# Autodesk Inventor assembly: !Clamp
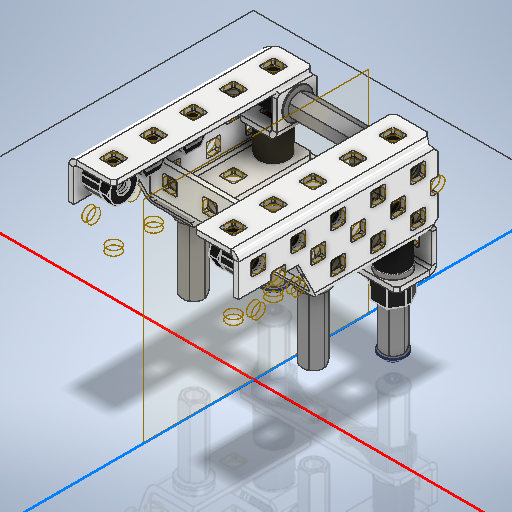
[picture p0: Inventor's stored thumbnail of the model, 512x512]
Saved by Autodesk Inventor 2026 (Build 300175000, 175)
## iProperties
Created: 2025-04-05
Part Number: !Clamp
Document SubType Name: Assembly
Designer: avere
Author: avere
## Documents named in this file (22)
- C:\Users\avere\OneDrive\Documents\VEX-CAD\V5-CAD\Clamp\!Clamp.iam
- C:\Users\avere\OneDrive\Documents\VEX-CAD\VEX-CAD-Inventor\Structure\C Channel\Aluminum 1x2x1\Alu C 1x2x1x5.ipt
- C:\Users\avere\OneDrive\Documents\VEX-CAD\VEX-CAD-Inventor\Motion\Shaft LS\Bearing Flat Low Profile.ipt
- C:\Users\avere\OneDrive\Documents\VEX-CAD\VEX-CAD-Inventor\Structure\Hardware\Nut Nylon\Nut Nylon - Black.ipt
- C:\Users\avere\OneDrive\Documents\VEX-CAD\VEX-CAD-Inventor\Structure\Hardware\Nut Nylon.ipt
- C:\Users\avere\OneDrive\Documents\VEX-CAD\VEX-CAD-Inventor\Structure\Standoff\Standoff .875.ipt
- C:\Users\avere\OneDrive\Documents\VEX-CAD\VEX-CAD-Inventor\Structure\Standoff.ipt
- C:\Users\avere\OneDrive\Documents\VEX-CAD\VEX-CAD-Inventor\Motion\Spacers\Spacer Nylon .375 OD\NSpacer .375 OD x .375.ipt
- C:\Users\avere\OneDrive\Documents\VEX-CAD\VEX-CAD-Inventor\Motion\Spacers\Spacer Nylon .375 OD.ipt
- C:\Users\avere\OneDrive\Documents\VEX-CAD\VEX-CAD-Inventor\Motion\Spacers\Washer Steel\SWasher .375 OD x .062500.ipt
- C:\Users\avere\OneDrive\Documents\VEX-CAD\VEX-CAD-Inventor\Motion\Spacers\Washer Steel.ipt
- C:\Users\avere\OneDrive\Documents\VEX-CAD\VEX-CAD-Inventor\Motion\Spacers\Washer Steel\SWasher .375 OD x .031250.ipt
- C:\Users\avere\OneDrive\Documents\VEX-CAD\VEX-CAD-Inventor\Structure\1-Post Standoff Retainer.ipt
- C:\Users\avere\OneDrive\Documents\VEX-CAD\VEX-CAD-Inventor\Structure\Standoff\Standoff .75.ipt
- C:\Users\avere\OneDrive\Documents\VEX-CAD\VEX-CAD-Inventor\Structure\Hardware\Screw Steel - Star\SScrew Star Smooth .250.ipt
- C:\Users\avere\OneDrive\Documents\VEX-CAD\VEX-CAD-Inventor\Structure\Hardware\Screw Steel - Star.ipt
- C:\Users\avere\OneDrive\Documents\VEX-CAD\VEX-CAD-Inventor\Structure\Angle\Aluminum 1x1\Alu Angle 1x1x1.ipt
- C:\Users\avere\OneDrive\Documents\VEX-CAD\VEX-CAD-Inventor\Motion\Spacers\Washer Steel\SWasher .375 OD x .015625.ipt
- C:\Users\avere\OneDrive\Documents\VEX-CAD\VEX-CAD-Inventor\Motion\Spacers\Washer Teflon\TWasher .375 OD x .04000.ipt
- C:\Users\avere\OneDrive\Documents\VEX-CAD\VEX-CAD-Inventor\Motion\Spacers\Washer Teflon.ipt
- C:\Users\avere\OneDrive\Documents\VEX-CAD\VEX-CAD-Inventor\Structure\C Channel\Aluminum 1x2x1\Alu C 1x2x1x5 Mirrored.ipt
- C:\Users\avere\OneDrive\Documents\VEX-CAD\VEX-CAD-Inventor\Structure\Angle\Aluminum 1x1\Alu Angle 1x1x4.ipt
## Components (41 placed, 15 different names)
1. Alu C 1x2x1x5:1 — Flush:1, Mate:1, Flush:2, Insert:1, Mate:2, Insert:5, Insert:8, Mate:3, Mate:4, Insert:13, Insert:37
2. Bearing Flat Low Profile:1 — Insert:1, Mate:2, Insert:2
3. Nut Nylon - Black:1 — Insert:2
4. Standoff .875:1 — Insert:7
5. NSpacer .375 OD x .375:1 — Insert:4, Insert:5
6. SWasher .375 OD x .062500:1 — Insert:4, Insert:9, Insert:36
7. SWasher .375 OD x .031250:2 — Insert:6, Insert:7
8. SWasher .375 OD x .062500:3 — Insert:6, Insert:8
9. 1-Post Standoff Retainer:1 — Insert:9, Insert:11
10. Standoff .75:2 — Insert:10, Insert:11
11. SScrew Star Smooth .250:1 — Insert:10
12. Alu Angle 1x1x1:1 — Mate:3, Mate:4, Insert:17
13. NSpacer .375 OD x .375:2 — Insert:12, Insert:13
14. SWasher .375 OD x .015625:4 — Insert:12
15. NSpacer .375 OD x .375:3 — Insert:16, Insert:17
16. TWasher .375 OD x .04000:1 — Insert:14, Insert:15
17. TWasher .375 OD x .04000:2 — Insert:14, Insert:16
18. SWasher .375 OD x .031250:5 — Insert:15
19. Alu C 1x2x1x5 Mirrored:1 — Flush:3, Mate:5, Flush:4, Mate:6, Insert:19, Insert:21, Insert:24, Mate:7, Mate:8, Insert:29, Mate:10
20. Bearing Flat Low Profile:2 — Mate:6, Insert:19, Insert:20
21. Nut Nylon - Black:2 — Insert:20
22. Standoff .875:3 — Insert:23
23. NSpacer .375 OD x .375:4 — Insert:21, Insert:22
24. SWasher .375 OD x .062500:6 — Insert:22, Insert:26, Mate:9
25. SWasher .375 OD x .031250:7 — Insert:23, Insert:25
26. SWasher .375 OD x .062500:8 — Insert:24, Insert:25
27. 1-Post Standoff Retainer:2 — Insert:26, Insert:27
28. Standoff .75:4 — Insert:27, Insert:28
29. SScrew Star Smooth .250:2 — Insert:28
30. Alu Angle 1x1x1:2 — Mate:7, Mate:8, Insert:31, Insert:40
31. NSpacer .375 OD x .375:5 — Insert:29, Insert:30
32. SWasher .375 OD x .015625:9 — Insert:30
33. NSpacer .375 OD x .375:6 — Insert:31, Insert:32
34. TWasher .375 OD x .04000:3 — Insert:33, Insert:34
35. TWasher .375 OD x .04000:4 — Insert:32, Insert:33
36. SWasher .375 OD x .031250:10 — Insert:34
37. Alu Angle 1x1x4:1 — Insert:36, Mate:9
38. Alu Angle 1x1x4:2 — Insert:37, Mate:10
39. Standoff .875:5 — Insert:38, Insert:39
40. SWasher .375 OD x .015625:11 — Insert:39
41. SWasher .375 OD x .015625:12 — Insert:38, Insert:40
## Relationships (51: Insert 37, Mate 10, Flush 4)
- Flush:1 (-31.75 mm): Alu C 1x2x1x5:1
- Mate:1 (19.05 mm): Alu C 1x2x1x5:1
- Flush:2 (-12.7 mm): Alu C 1x2x1x5:1
- Insert:1: Alu C 1x2x1x5:1 ↔ Bearing Flat Low Profile:1
- Mate:2: Alu C 1x2x1x5:1 ↔ Bearing Flat Low Profile:1
- Insert:2 (1.27 mm): Bearing Flat Low Profile:1 ↔ Nut Nylon - Black:1
- Insert:4: NSpacer .375 OD x .375:1 ↔ SWasher .375 OD x .062500:1
- Insert:5: Alu C 1x2x1x5:1 ↔ NSpacer .375 OD x .375:1
- Insert:6: SWasher .375 OD x .031250:2 ↔ SWasher .375 OD x .062500:3
- Insert:7: Standoff .875:1 ↔ SWasher .375 OD x .031250:2
- Insert:8: Alu C 1x2x1x5:1 ↔ SWasher .375 OD x .062500:3
- Insert:9 (1.5875 mm): SWasher .375 OD x .062500:1 ↔ 1-Post Standoff Retainer:1
- Insert:10: Standoff .75:2 ↔ SScrew Star Smooth .250:1
- Insert:11: 1-Post Standoff Retainer:1 ↔ Standoff .75:2
- Mate:3: Alu C 1x2x1x5:1 ↔ Alu Angle 1x1x1:1
- Mate:4: Alu C 1x2x1x5:1 ↔ Alu Angle 1x1x1:1
- Insert:12: NSpacer .375 OD x .375:2 ↔ SWasher .375 OD x .015625:4
- Insert:13: Alu C 1x2x1x5:1 ↔ NSpacer .375 OD x .375:2
- Insert:14: TWasher .375 OD x .04000:1 ↔ TWasher .375 OD x .04000:2
- Insert:15: TWasher .375 OD x .04000:1 ↔ SWasher .375 OD x .031250:5
- Insert:16: NSpacer .375 OD x .375:3 ↔ TWasher .375 OD x .04000:2
- Insert:17: Alu Angle 1x1x1:1 ↔ NSpacer .375 OD x .375:3
- Flush:3 (-12.7 mm): Alu C 1x2x1x5 Mirrored:1
- Mate:5 (-19.05 mm): Alu C 1x2x1x5 Mirrored:1
- Flush:4 (-31.75 mm): Alu C 1x2x1x5 Mirrored:1
- Mate:6: Alu C 1x2x1x5 Mirrored:1 ↔ Bearing Flat Low Profile:2
- Insert:19: Alu C 1x2x1x5 Mirrored:1 ↔ Bearing Flat Low Profile:2
- Insert:20 (1.27 mm): Bearing Flat Low Profile:2 ↔ Nut Nylon - Black:2
- Insert:21: Alu C 1x2x1x5 Mirrored:1 ↔ NSpacer .375 OD x .375:4
- Insert:22: NSpacer .375 OD x .375:4 ↔ SWasher .375 OD x .062500:6
- Insert:23: Standoff .875:3 ↔ SWasher .375 OD x .031250:7
- Insert:24: Alu C 1x2x1x5 Mirrored:1 ↔ SWasher .375 OD x .062500:8
- Insert:25: SWasher .375 OD x .031250:7 ↔ SWasher .375 OD x .062500:8
- Insert:26 (1.5875 mm): SWasher .375 OD x .062500:6 ↔ 1-Post Standoff Retainer:2
- Insert:27: 1-Post Standoff Retainer:2 ↔ Standoff .75:4
- Insert:28: Standoff .75:4 ↔ SScrew Star Smooth .250:2
- Mate:7: Alu C 1x2x1x5 Mirrored:1 ↔ Alu Angle 1x1x1:2
- Mate:8: Alu C 1x2x1x5 Mirrored:1 ↔ Alu Angle 1x1x1:2
- Insert:29: Alu C 1x2x1x5 Mirrored:1 ↔ NSpacer .375 OD x .375:5
- Insert:30: NSpacer .375 OD x .375:5 ↔ SWasher .375 OD x .015625:9
- Insert:31: Alu Angle 1x1x1:2 ↔ NSpacer .375 OD x .375:6
- Insert:32: NSpacer .375 OD x .375:6 ↔ TWasher .375 OD x .04000:4
- Insert:33: TWasher .375 OD x .04000:3 ↔ TWasher .375 OD x .04000:4
- Insert:34: TWasher .375 OD x .04000:3 ↔ SWasher .375 OD x .031250:10
- Insert:36: SWasher .375 OD x .062500:1 ↔ Alu Angle 1x1x4:1
- Mate:9: SWasher .375 OD x .062500:6 ↔ Alu Angle 1x1x4:1
- Insert:37: Alu C 1x2x1x5:1 ↔ Alu Angle 1x1x4:2
- Mate:10: Alu C 1x2x1x5 Mirrored:1 ↔ Alu Angle 1x1x4:2
- Insert:38: Standoff .875:5 ↔ SWasher .375 OD x .015625:12
- Insert:39: Standoff .875:5 ↔ SWasher .375 OD x .015625:11
- Insert:40: Alu Angle 1x1x1:2 ↔ SWasher .375 OD x .015625:12
